# Autodesk Inventor assembly: Shape Strip Test
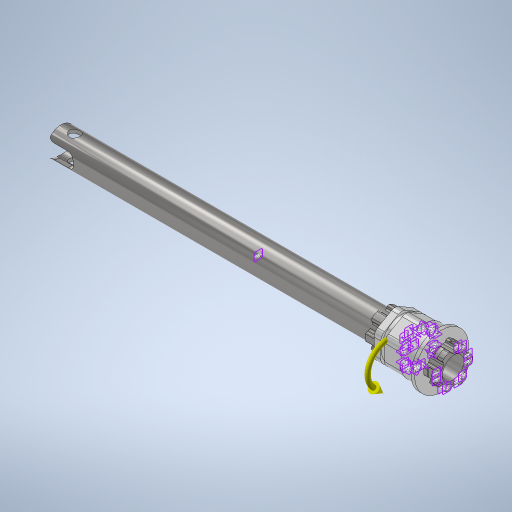
[picture p0: Inventor's stored thumbnail of the model, 512x512]
Saved by Autodesk Inventor 2023.2 (Build 272271000, 271)
## iProperties
Created: 2024-01-31
Part Number: Shape Strip Test
Document SubType Name: Assembly
Designer: Nathan Cai
Author: Nathan Cai
## Documents named in this file (9)
- E:\Documents\Inventor\Misc\Shape Strip Test.iam
- E:\Documents\Inventor\Misc\Bushing.ipt
- E:\Documents\Inventor\Misc\Shaft.ipt
- E:\Documents\Inventor\Misc\Shape Strip Test\AIP\FEA\elf30vqu8.fins
- E:\Documents\Inventor\Misc\Shape Strip Test\AIP\FEA\elf30vqu8.fsat
- E:\Documents\Inventor\Misc\Shape Strip Test\AIP\FEA\elf30vqu8.ftes
- E:\Documents\Inventor\Misc\Shape Strip Test\AIP\FEA\elf30vqu8.fwiz
- E:\Documents\Inventor\Misc\Shape Strip Test\AIP\FEA\elf30vqww.fmsh
- E:\Documents\Inventor\Misc\Shape Strip Test\AIP\FEA\elf30vqwx.fres
## Components (2 placed, 2 different names)
1. Bushing:1 — Mate:1, Mate:2, Flush:1
2. Shaft:1 — Mate:1, Mate:2, Flush:1
## Relationships (3: Mate 2, Flush 1)
- Mate:1: Bushing:1 ↔ Shaft:1
- Mate:2: Bushing:1 ↔ Shaft:1
- Flush:1 (1 mm): Bushing:1 ↔ Shaft:1
## Named parameters: sa_0 = 11298.5
note: some values were not read from the file. Shown as the stored number, unit unknown: "sa_0".
